# Autodesk Inventor assembly: Elektro_asm
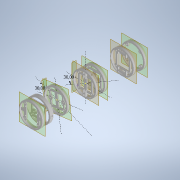
[picture p0: Inventor's stored thumbnail of the model, 180x180]
Saved by Autodesk Inventor 2020 (Build 240168000, 168)
## iProperties
Created: 2022-03-10
Part Number: Elektro_asm
Document SubType Name: Assembly
Designer: sp
Author: sp
## Documents named in this file (8)
- C:\Users\sp\Documents\Rocket\rocket\CAD\Elektro_asm.iam
- C:\Users\sp\Documents\Rocket\rocket\CAD\Electro_unit.ipt
- C:\Users\sp\Documents\Rocket\rocket\CAD\Elektro_Gyro.ipt
- C:\Users\sp\Documents\Rocket\rocket\CAD\Electro_gps.ipt
- C:\Users\sp\Documents\Rocket\rocket\CAD\Electro_bat_down.ipt
- C:\Users\sp\Documents\Rocket\rocket\CAD\Electro_bat_up.ipt
- C:\Users\sp\Documents\Rocket\rocket\CAD\Electro_esp32.ipt
- C:\Users\sp\Documents\Rocket\rocket\CAD\Electro_esp32_up.ipt
## Components (7 placed, 7 different names)
1. Electro_unit:1 — Einfügen:5, Passend:1
2. Elektro_Gyro:1 — Einfügen:3, Einfügen:4
3. Electro_gps:1 — Einfügen:3
4. Electro_bat_down:1 — Einfügen:4, Einfügen:6, Einfügen:8, Passend:2, Passend:3
5. Electro_bat_up:1 — Einfügen:5, Einfügen:8, Passend:1, Passend:2
6. Electro_esp32:1 — Einfügen:6, Passend:3, Einfügen:9
7. Electro_esp32_up:1 — Einfügen:9
## Relationships (9: Insert 6, Mate 3)
- Einfügen:3 [Insert] (10 mm): Elektro_Gyro:1 ↔ Electro_gps:1
- Einfügen:4 [Insert] (130 mm): Elektro_Gyro:1 ↔ Electro_bat_down:1
- Einfügen:5 [Insert] (20 mm): Electro_unit:1 ↔ Electro_bat_up:1
- Einfügen:6 [Insert] (15 mm): Electro_bat_down:1 ↔ Electro_esp32:1
- Einfügen:8 [Insert] (65 mm): Electro_bat_down:1 ↔ Electro_bat_up:1
- Passend:1 [Mate]: Electro_unit:1 ↔ Electro_bat_up:1
- Passend:2 [Mate]: Electro_bat_down:1 ↔ Electro_bat_up:1
- Passend:3 [Mate]: Electro_bat_down:1 ↔ Electro_esp32:1
- Einfügen:9 [Insert] (65 mm): Electro_esp32:1 ↔ Electro_esp32_up:1
